# Autodesk Inventor assembly: DribblerUnit
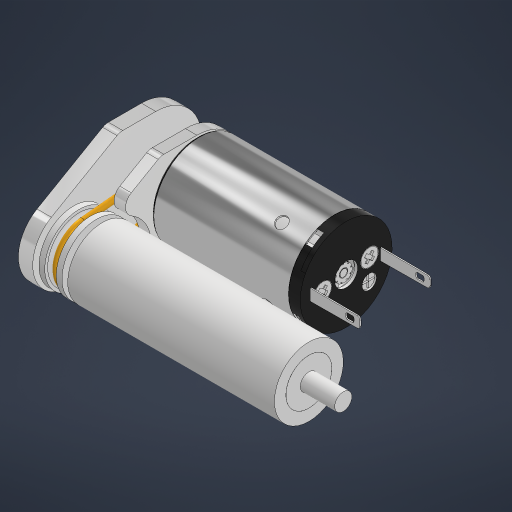
[picture p0: Inventor's stored thumbnail of the model, 512x512]
Saved by Autodesk Inventor 2024.2 (Build 282272000, 272)
## iProperties
Created: 2023-12-27
Part Number: DribblerUnit
Document SubType Name: Assembly
Designer: Hanaoka
Author: Hanaoka
## Documents named in this file (11)
- G:\共有ドライブ\reRo\05_個人\hanaoka\inventor\DribblerUnit\DribblerUnit.iam
- G:\共有ドライブ\reRo\05_個人\hanaoka\inventor\DribblerUnit\Dribbler_Tube.ipt
- G:\共有ドライブ\reRo\05_個人\hanaoka\inventor\DribblerUnit\Shaft_350.ipt
- G:\共有ドライブ\reRo\05_個人\hanaoka\inventor\DribblerUnit\Bearing_C-FL673ZZ\Bearing_C-FL673ZZ.ipt
- G:\共有ドライブ\reRo\05_個人\hanaoka\inventor\DribblerUnit\Tube_Hub.ipt
- G:\共有ドライブ\reRo\05_個人\hanaoka\inventor\DribblerUnit\Althonix16dct\Althonix16dct.ipt
- G:\共有ドライブ\reRo\05_個人\hanaoka\inventor\HandleUnit\GearCover.ipt
- G:\共有ドライブ\reRo\05_個人\hanaoka\inventor\Spacer\Pulley_Small.ipt
- G:\共有ドライブ\reRo\05_個人\hanaoka\inventor\Spacer\Pulley_Big.ipt
- G:\共有ドライブ\reRo\05_個人\hanaoka\inventor\PCBs\Motor_Mount.ipt
- G:\共有ドライブ\reRo\05_個人\hanaoka\inventor\PCBs\Belt.ipt
## Components (10 placed, 10 different names)
1. Dribbler_Tube:1 — 挿入:12
2. Shaft_350:1 — 挿入:1, 挿入:10, 挿入:13
3. Bearing_C-FL673ZZ:1 — 挿入:1, 挿入:6
4. Tube_Hub:1 — 挿入:12, 挿入:13
5. Althonix16dct:1 — 挿入:9, 挿入:11, メイト:1
6. GearCover:1 — 挿入:6
7. Pulley_Small:1 — 挿入:9
8. Pulley_Big:1 — 挿入:10
9. Motor_Mount:1 — 挿入:11, メイト:1
10. Belt:1
## Relationships (8: Insert 7, Mate 1)
- 挿入:1 [Insert]: Shaft_350:1 ↔ Bearing_C-FL673ZZ:1
- 挿入:6 [Insert]: Bearing_C-FL673ZZ:1 ↔ GearCover:1
- 挿入:9 [Insert] (1 mm): Althonix16dct:1 ↔ Pulley_Small:1
- 挿入:10 [Insert] (3 mm): Shaft_350:1 ↔ Pulley_Big:1
- 挿入:11 [Insert]: Althonix16dct:1 ↔ Motor_Mount:1
- メイト:1 [Mate]: Althonix16dct:1 ↔ Motor_Mount:1
- 挿入:12 [Insert]: Dribbler_Tube:1 ↔ Tube_Hub:1
- 挿入:13 [Insert] (8 mm): Shaft_350:1 ↔ Tube_Hub:1
